# Autodesk Inventor assembly: сборка захвата
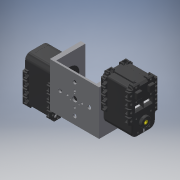
[picture p0: Inventor's stored thumbnail of the model, 180x180]
Saved by Autodesk Inventor 2019 (Build 230136000, 136)
## iProperties
Created: 2019-08-15
Part Number: сборка захвата
Material: Типовые
Document SubType Name: Assembly
Designer: Петров Иван
Author: Петров Иван
## Documents named in this file (3)
- E:\IVAN\Kvantoriada2019\optimal_gripper\hardware\Стандартные изделия\Концевик механический\клешня\сборка захвата.iam
- E:\IVAN\Kvantoriada2019\optimal_gripper\hardware\Стандартные изделия\Концевик механический\клешня\база захвата.ipt
- E:\IVAN\Kvantoriada2019\optimal_gripper\hardware\Стандартные изделия\Сервомотор Dynamixel AX-12A\ax-12a.iam
## Components (3 placed, 2 different names)
1. база захвата:1 — Совмещение:1, Совмещение:2, Совмещение:3, Совмещение:4, Совмещение:5, Совмещение:6
2. ax-12a:1 [sub-assembly] — Совмещение:1, Совмещение:2, Совмещение:3
3. ax-12a:2 [sub-assembly] — Совмещение:4, Совмещение:5, Совмещение:6
## Relationships (6: Mate 6)
- Совмещение:1 [Mate]: база захвата:1 ↔ ax-12a:1
- Совмещение:2 [Mate]: база захвата:1 ↔ ax-12a:1
- Совмещение:3 [Mate]: база захвата:1 ↔ ax-12a:1
- Совмещение:4 [Mate]: база захвата:1 ↔ ax-12a:2
- Совмещение:5 [Mate]: база захвата:1 ↔ ax-12a:2
- Совмещение:6 [Mate]: база захвата:1 ↔ ax-12a:2
